# Autodesk Inventor assembly: Montagem_Motororreia e suporte
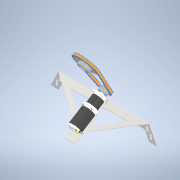
[picture p0: Inventor's stored thumbnail of the model, 180x180]
Saved by Autodesk Inventor 2022 (Build 260153000, 153)
## iProperties
Created: 2021-09-23
Part Number: Montagem_Motororreia e suporte
Document SubType Name: Assembly
Designer: Alison
Author: Alison
## Documents named in this file (4)
- C:\Users\Alison\Documents\TCC\Peças e desenho no inventor - TCC\Peças\Montagem_Motororreia e suporte.iam
- C:\Users\Alison\Documents\TCC\Desenhos e Montagem\Suporte para o motor e redutor1.ipt
- C:\Users\Alison\Downloads\23HS22-2804S-HG5.ipt
- C:\Users\Alison\Documents\TCC\Desenhos e Montagem\Montagem corrente.ipt
## Components (3 placed, 3 different names)
1. Suporte para o motor e redutor1:1 — Coincidente:2
2. 23HS22-2804S-HG5:1 — Coincidente:2, Coincidente:3
3. Montagem corrente:1 — Coincidente:3
## Relationships (2: Mate 2)
- Coincidente:2 [Mate]: Suporte para o motor e redutor1:1 ↔ 23HS22-2804S-HG5:1
- Coincidente:3 [Mate]: 23HS22-2804S-HG5:1 ↔ Montagem corrente:1
